# Autodesk Inventor assembly: test 3
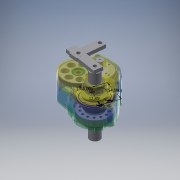
[picture p0: Inventor's stored thumbnail of the model, 180x180]
Saved by Autodesk Inventor 2018.1 (Build 221171000, 171)
## iProperties
Created: 2022-07-21
Part Number: test 3
Document SubType Name: Assembly
Designer: Bureau
Author: Bureau
## Documents named in this file (5)
- C:\Users\mouta\GoogleDrive\Manu\USINAGE\MoteurVelo\test 3.iam
- C:\Users\mouta\GoogleDrive\Manu\USINAGE\MoteurVelo\Corps\body gauche.ipt
- C:\Users\mouta\GoogleDrive\Manu\USINAGE\MoteurVelo\Assembly4.iam
- C:\Users\mouta\GoogleDrive\Manu\USINAGE\MoteurVelo\Corps\body milieu.ipt
- C:\Users\mouta\GoogleDrive\Manu\USINAGE\MoteurVelo\Corps\body droit bis.ipt
## Components (4 placed, 4 different names)
1. body gauche:1 — Mate:1, Flush:1, Mate:2, Mate:3, Mate:4
2. Assembly4:1 [sub-assembly] — Mate:1, Flush:1
3. body milieu:1 — Mate:2, Mate:3, Mate:4, Mate:5, Mate:6, Mate:7
4. body droit bis:1 — Mate:5, Mate:6, Mate:7
## Relationships (8: Mate 7, Flush 1)
- Mate:1: body gauche:1 ↔ Assembly4:1
- Flush:1 (-41 mm): body gauche:1 ↔ Assembly4:1
- Mate:2: body gauche:1 ↔ body milieu:1
- Mate:3: body gauche:1 ↔ body milieu:1
- Mate:4: body gauche:1 ↔ body milieu:1
- Mate:5: body milieu:1 ↔ body droit bis:1
- Mate:6: body milieu:1 ↔ body droit bis:1
- Mate:7: body milieu:1 ↔ body droit bis:1
